# Autodesk Inventor assembly: WRO FE vehicle v4.1
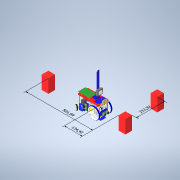
[picture p0: Inventor's stored thumbnail of the model, 180x180]
Saved by Autodesk Inventor 2022.6 (Build 266554000, 554)
## iProperties
Created: 2024-10-12
Part Number: WRO FE vehicle v4.1
Document SubType Name: Assembly
Designer: Zhong
Author: Zhong
## Documents named in this file (41)
- C:\Users\Zhong\Desktop\SP\YR_3_SEM_1\WRO\Robot\vehicle v8.4\WRO FE vehicle v8.iam
- C:\Users\Zhong\Desktop\SP\YR_3_SEM_1\WRO\Robot\vehicle v8.4\rear wheel 86mm.ipt
- C:\Users\Zhong\Desktop\SP\YR_3_SEM_1\WRO\Robot\vehicle v8.4\dfifferential.ipt
- C:\Users\Zhong\Desktop\SP\YR_3_SEM_1\WRO\Robot\vehicle v8.4\rear shaft v2.ipt
- rear shaft.ipt
- C:\Users\Zhong\Desktop\SP\YR_3_SEM_1\WRO\Robot\vehicle v8.4\Bottom plate.ipt
- C:\Users\Zhong\Desktop\SP\YR_3_SEM_1\WRO\Robot\vehicle v8.4\motor_small.ipt
- C:\Users\Zhong\Desktop\SP\YR_3_SEM_1\WRO\Robot\vehicle v8.4\driver gear adapter v2.ipt
- C:\Users\Zhong\Desktop\SP\YR_3_SEM_1\WRO\Robot\vehicle v8.4\DC+bearing mount.ipt
- C:\Users\Zhong\Desktop\SP\YR_3_SEM_1\WRO\Robot\vehicle v8.4\new battery.ipt
- C:\Users\Zhong\Desktop\SP\YR_3_SEM_1\WRO\Robot\vehicle v8.4\servo motor HS-7955TG.iam
- C:\Users\Zhong\Desktop\SP\YR_3_SEM_1\WRO\Robot\vehicle v8.4\US-015.ipt
- C:\Users\Zhong\Desktop\SP\YR_3_SEM_1\WRO\Robot\vehicle v8.4\stand M3-L30.ipt
- C:\Users\Zhong\Desktop\SP\YR_3_SEM_1\WRO\Robot\vehicle v8.4\Top plate.ipt
- C:\Users\Zhong\Desktop\SP\YR_3_SEM_1\WRO\Robot\vehicle v8.4\stand M3-L10.ipt
- C:\Users\Zhong\Desktop\SP\YR_3_SEM_1\WRO\Robot\vehicle v8.4\raspberry pi.ipt
- C:\Users\Zhong\Desktop\SP\YR_3_SEM_1\WRO\Robot\vehicle v8.4\Vertical Ultrasonic Sensor Mount.ipt
- C:\Users\Zhong\Desktop\SP\YR_3_SEM_1\WRO\Robot\vehicle v8.4\ultrasonic and headlight mount.ipt
- C:\Users\Zhong\Desktop\SP\YR_3_SEM_1\WRO\Robot\vehicle v8.4\MainLink.ipt
- C:\Users\Zhong\Desktop\SP\YR_3_SEM_1\WRO\Robot\vehicle v8.4\ActuatorLink.ipt
- C:\Users\Zhong\Desktop\SP\YR_3_SEM_1\WRO\Robot\vehicle v8.4\Battery Mount V2.ipt
- C:\Users\Zhong\Desktop\SP\YR_3_SEM_1\WRO\Robot\vehicle v8.4\Wheel_Pivot.ipt
- C:\Users\Zhong\Desktop\SP\YR_3_SEM_1\WRO\Robot\vehicle v8.4\LM2596 Buck Converter.ipt
- C:\Users\Zhong\Desktop\SP\YR_3_SEM_1\WRO\Robot\vehicle v8.4\LED Light.ipt
- C:\Users\Zhong\Desktop\SP\YR_3_SEM_1\WRO\Robot\vehicle v8.4\front wheel v2.ipt
- C:\Users\Zhong\Desktop\SP\YR_3_SEM_1\WRO\Robot\vehicle v8.4\front wheel mount.ipt
- C:\Users\Zhong\Desktop\SP\YR_3_SEM_1\WRO\Robot\vehicle v8.4\camera mount+HMC angled.ipt
- C:\Users\Zhong\Desktop\SP\YR_3_SEM_1\WRO\Robot\vehicle v8.4\Obstacle.ipt
- C:\Users\Zhong\Desktop\SP\YR_3_SEM_1\WRO\Robot\vehicle v8.4\cam vision.ipt
- C:\Users\Zhong\Desktop\SP\YR_3_SEM_1\WRO\Robot\vehicle v8.4\stand M3-L5.ipt
- C:\Users\Zhong\Desktop\SP\YR_3_SEM_1\WRO\Robot\vehicle v8.4\Servo steering actuator.ipt
- C:\Users\Zhong\Desktop\SP\YR_3_SEM_1\WRO\Robot\vehicle v8.4\Servo mount.ipt
- C:\Users\Zhong\Desktop\SP\YR_3_SEM_1\WRO\Robot\vehicle v8.4\Servo mount Right.ipt
- C:\Users\Zhong\Desktop\SP\YR_3_SEM_1\WRO\Robot\vehicle v8.4\Servo steering actuator v2.ipt
- C:\Users\Zhong\Desktop\SP\YR_3_SEM_1\WRO\Robot\vehicle v8.4\Vertical TOF mount.ipt
- C:\Users\Zhong\Desktop\SP\YR_3_SEM_1\WRO\Robot\vehicle v8.4\stand M3-L7.ipt
- C:\Users\Zhong\Desktop\SP\YR_3_SEM_1\WRO\Robot\vehicle v8.4\camera mount.ipt
- C:\Users\Zhong\Desktop\SP\YR_3_SEM_1\WRO\Robot\vehicle v8.4\IMU mount.ipt
- C:\Users\Zhong\Desktop\SP\YR_3_SEM_1\WRO\Robot\vehicle v8.4\front TOF mount.ipt
- C:\Users\Zhong\Desktop\SP\YR_3_SEM_1\WRO\Robot\vehicle v8.4\camera+light+IMU.ipt
- C:\Users\Zhong\Desktop\SP\YR_3_SEM_1\WRO\Robot\vehicle v8.4\cam mount prototype.ipt
## Components (74 placed, 39 different names)
1. rear wheel 86mm:1 — Tangent:2, Insert:4, Symmetry:1
2. rear wheel 86mm:2 — Tangent:1, Insert:2, Symmetry:1
3. dfifferential:1 — Angle:4, Insert:1, Insert:3
4. rear shaft:1 — Insert:3, Insert:4, Mate:20
5. rear shaft:2 — Insert:1, Insert:2
6. Bottom plate:1 — Flush:1, Tangent:3, Angle:5, Flush:2, Mate:1, Mate:2, Mate:3, Insert:17, Insert:18, Mate:95, Insert:21, Insert:22, Insert:23, Insert:24, Mate:108, Insert:71, Insert:72, Mate:110, Insert:75, Mate:112, Insert:77, Insert:78, Mate:113, Insert:87, Insert:89, Insert:94, Insert:95, Insert:96, Insert:97, Insert:98, Mate:116, Mate:117, Insert:101, Flush:116, Mate:124, Flush:117, Mate:125
7. motor_small:1 — Tangent:3, Flush:2, Insert:14, Insert:123
8. driver gear adapter v2:1 — Insert:123
9. DC+bearing mount:1 — Mate:1, Mate:2, Mate:3, Mate:20, Insert:14
10. new battery:1 — Mate:119, Mate:120, Mate:121
11. servo motor HS-7955TG:1 [sub-assembly] — Mate:95, Mate:110, Mate:113, Insert:80, Mate:114, Insert:85, Insert:86, Insert:92, Insert:93, Insert:126
12. US-015:1 — Insert:15, Insert:16
13. Top plate:1 — Insert:49, Insert:50, Insert:55, Insert:56, Insert:57, Insert:59, Insert:60, Insert:79, Insert:102, Insert:103, Insert:108, Insert:109, Mate:123, Insert:119, Insert:120
14. raspberry pi:1 — Insert:45, Insert:46, Insert:47, Insert:48
15. Vertical Ultrasonic Sensor Mount:1 — Mate:64, Mate:65, Mate:66, Insert:21, Insert:22
16. Vertical Ultrasonic Sensor Mount:2 — Mate:61, Mate:62, Mate:63, Insert:23, Insert:24
17. US-015:2 — Mate:64, Mate:65, Mate:66
18. US-015:3 — Mate:61, Mate:62, Mate:63
19. ultrasonic and headlight mount:1 — Insert:15, Insert:16, Insert:17, Insert:18
20. MainLink:1 — Mate:102, Insert:77, Insert:78, Angle:6
21. ActuatorLink:1 — Mate:97, Mate:99, Angle:6, Tangent:6, Insert:99, Insert:100, Tangent:7
22. Wheel_Pivot:1 — Mate:97, Insert:82, Insert:97, Insert:100
23. Wheel_Pivot:2 — Mate:99, Mate:102, Insert:81, Insert:98, Insert:99
24. LED Light:1 — Mate:122, Insert:135
25. front wheel v2:1 — Tangent:4, Insert:83, Flush:115
26. front wheel v2:2 — Flush:112, Tangent:5, Insert:84
27. front wheel mount:1 — Flush:112, Mate:112, Insert:81, Insert:84
28. stand M3-L10:13 — Insert:117
29. stand M3-L10:14 — Insert:44, Insert:116
30. stand M3-L10:15 — Insert:118
31. stand M3-L10:16 — Insert:112, Insert:115
32. Obstacle:1 — Mate:107, Mate:108, Flush:118, Flush:119
33. cam vision:1 — Insert:44, Insert:112, Insert:127, Insert:128
34. stand M3-L10:17 — Insert:48
35. stand M3-L10:18 — Insert:46, Insert:50
36. stand M3-L10:19 — Insert:47
37. stand M3-L10:20 — Insert:45, Insert:49
38. stand M3-L5:1 — Insert:56, Insert:113, Insert:129
39. stand M3-L5:2
40. stand M3-L5:3
41. stand M3-L5:4 — Insert:55, Insert:114, Insert:130
42. stand M3-L5:5 — Insert:79
43. stand M3-L5:6 — Insert:59, Insert:61
44. stand M3-L5:7 — Insert:60
45. stand M3-L5:8 — Insert:57, Insert:62
46. LM2596 Buck Converter:1 — Insert:61, Insert:62
47. stand M3-L30:1 — Insert:66, Insert:122
48. stand M3-L30:2 — Insert:66
49. stand M3-L30:3 — Insert:65, Insert:121
50. stand M3-L30:4 — Insert:65, Insert:72
51. stand M3-L30:5 — Insert:64, Insert:71
52. stand M3-L30:6 — Insert:64, Insert:104
53. stand M3-L30:7 — Insert:63, Insert:105
54. stand M3-L30:8 — Insert:63, Insert:75
55. Servo steering actuator:1 — Tangent:6, Insert:80
56. front wheel mount:2 — Insert:82, Insert:83, Flush:115
57. Servo mount:1 — Mate:114, Insert:85, Insert:86, Insert:87, Insert:89, Insert:101
58. Servo mount Right:1 — Insert:92, Insert:93, Insert:94, Insert:95, Insert:96
59. Servo steering actuator v2:1 — Mate:116, Insert:126, Tangent:7
60. Vertical TOF mount:1 — Mate:117, Flush:116
61. Battery Mount V2:1 — Insert:102, Insert:103, Mate:119, Mate:120, Mate:121
62. stand M3-L7:1 — Insert:104, Insert:108
63. stand M3-L7:2 — Insert:105, Insert:109
64. Obstacle:2 — Flush:119
65. camera mount+HMC angled:1 — Mate:122, Insert:113, Insert:114, Insert:135, Insert:136, Insert:137
66. camera mount:1 — Mate:123, Insert:115, Insert:116, Insert:117, Insert:118, Insert:119, Insert:120
67. stand M3-L5:9 — Insert:122
68. stand M3-L5:10 — Insert:121
69. IMU mount:1 — Insert:136, Insert:137
70. front TOF mount:1 — Mate:125
71. camera+light+IMU:1 — Insert:127, Insert:128, Insert:129, Insert:130
72. Obstacle:3 — Flush:118
73. cam mount prototype:1
74. Vertical TOF mount:2 — Mate:124, Flush:117
## Relationships (131: Insert 82, Mate 29, Flush 8, Tangent 7, Angle 4, Symmetry 1)
- Tangent:1: rear wheel 86mm:2
- Angle:2 (0 deg)
- Tangent:2: rear wheel 86mm:1
- Angle:4 (0 deg): dfifferential:1
- Insert:1: dfifferential:1 ↔ rear shaft:2
- Insert:2 (-2 mm): rear wheel 86mm:2 ↔ rear shaft:2
- Insert:3: dfifferential:1 ↔ rear shaft:1
- Insert:4 (-2 mm): rear wheel 86mm:1 ↔ rear shaft:1
- Flush:1: Bottom plate:1
- Symmetry:1: rear wheel 86mm:1 ↔ rear wheel 86mm:2
- Tangent:3 (6 mm): Bottom plate:1 ↔ motor_small:1
- Angle:5 (180 deg): Bottom plate:1
- Flush:2: Bottom plate:1 ↔ motor_small:1
- Mate:1: Bottom plate:1 ↔ DC+bearing mount:1
- Mate:2: Bottom plate:1 ↔ DC+bearing mount:1
- Mate:3: Bottom plate:1 ↔ DC+bearing mount:1
- Mate:20: rear shaft:1 ↔ DC+bearing mount:1
- Mate:61: Vertical Ultrasonic Sensor Mount:2 ↔ US-015:3
- Mate:62: Vertical Ultrasonic Sensor Mount:2 ↔ US-015:3
- Mate:63: Vertical Ultrasonic Sensor Mount:2 ↔ US-015:3
- Mate:64: Vertical Ultrasonic Sensor Mount:1 ↔ US-015:2
- Mate:65: Vertical Ultrasonic Sensor Mount:1 ↔ US-015:2
- Mate:66: Vertical Ultrasonic Sensor Mount:1 ↔ US-015:2
- Insert:14: motor_small:1 ↔ DC+bearing mount:1
- Insert:15: US-015:1 ↔ ultrasonic and headlight mount:1
- Insert:16: US-015:1 ↔ ultrasonic and headlight mount:1
- Insert:17: Bottom plate:1 ↔ ultrasonic and headlight mount:1
- Insert:18: Bottom plate:1 ↔ ultrasonic and headlight mount:1
- Mate:95: Bottom plate:1 ↔ servo motor HS-7955TG:1
- Mate:97: ActuatorLink:1 ↔ Wheel_Pivot:1
- Mate:99: ActuatorLink:1 ↔ Wheel_Pivot:2
- Mate:102: MainLink:1 ↔ Wheel_Pivot:2
- Insert:21: Bottom plate:1 ↔ Vertical Ultrasonic Sensor Mount:1
- Insert:22: Bottom plate:1 ↔ Vertical Ultrasonic Sensor Mount:1
- Insert:23: Bottom plate:1 ↔ Vertical Ultrasonic Sensor Mount:2
- Insert:24: Bottom plate:1 ↔ Vertical Ultrasonic Sensor Mount:2
- Flush:112: front wheel v2:2 ↔ front wheel mount:1
- Mate:107: Obstacle:1
- Mate:108: Bottom plate:1 ↔ Obstacle:1
- Insert:44: stand M3-L10:14 ↔ cam vision:1
- Insert:45: raspberry pi:1 ↔ stand M3-L10:20
- Insert:46: raspberry pi:1 ↔ stand M3-L10:18
- Insert:47: raspberry pi:1 ↔ stand M3-L10:19
- Insert:48: raspberry pi:1 ↔ stand M3-L10:17
- Insert:49: Top plate:1 ↔ stand M3-L10:20
- Insert:50: Top plate:1 ↔ stand M3-L10:18
- Insert:55: Top plate:1 ↔ stand M3-L5:4
- Insert:56: Top plate:1 ↔ stand M3-L5:1
- Insert:57: Top plate:1 ↔ stand M3-L5:8
- Insert:59: Top plate:1 ↔ stand M3-L5:6
- Insert:60: Top plate:1 ↔ stand M3-L5:7
- Insert:61: stand M3-L5:6 ↔ LM2596 Buck Converter:1
- Insert:62: stand M3-L5:8 ↔ LM2596 Buck Converter:1
- Insert:63: stand M3-L30:7 ↔ stand M3-L30:8
- Insert:64: stand M3-L30:5 ↔ stand M3-L30:6
- Insert:65: stand M3-L30:3 ↔ stand M3-L30:4
- Insert:66: stand M3-L30:1 ↔ stand M3-L30:2
- Insert:71: Bottom plate:1 ↔ stand M3-L30:5
- Insert:72: Bottom plate:1 ↔ stand M3-L30:4
- Mate:110: Bottom plate:1 ↔ servo motor HS-7955TG:1
- Insert:75: Bottom plate:1 ↔ stand M3-L30:8
- Tangent:4: front wheel v2:1
- Mate:112: Bottom plate:1 ↔ front wheel mount:1
- Tangent:5: front wheel v2:2
- Insert:77: Bottom plate:1 ↔ MainLink:1
- Insert:78: Bottom plate:1 ↔ MainLink:1
- Mate:113 (8 mm): Bottom plate:1 ↔ servo motor HS-7955TG:1
- Insert:79: Top plate:1 ↔ stand M3-L5:5
- Angle:6 (0 deg): MainLink:1 ↔ ActuatorLink:1
- Tangent:6: ActuatorLink:1 ↔ Servo steering actuator:1
- Insert:80 (2 mm): servo motor HS-7955TG:1 ↔ Servo steering actuator:1
- Insert:81: Wheel_Pivot:2 ↔ front wheel mount:1
- Insert:82: Wheel_Pivot:1 ↔ front wheel mount:2
- Insert:83 (1 mm): front wheel v2:1 ↔ front wheel mount:2
- Flush:115: front wheel v2:1 ↔ front wheel mount:2
- Insert:84: front wheel v2:2 ↔ front wheel mount:1
- Mate:114: servo motor HS-7955TG:1 ↔ Servo mount:1
- Insert:85: servo motor HS-7955TG:1 ↔ Servo mount:1
- Insert:86: servo motor HS-7955TG:1 ↔ Servo mount:1
- Insert:87: Bottom plate:1 ↔ Servo mount:1
- Insert:89: Bottom plate:1 ↔ Servo mount:1
- Insert:92: servo motor HS-7955TG:1 ↔ Servo mount Right:1
- Insert:93: servo motor HS-7955TG:1 ↔ Servo mount Right:1
- Insert:94: Bottom plate:1 ↔ Servo mount Right:1
- Insert:95: Bottom plate:1 ↔ Servo mount Right:1
- Insert:96: Bottom plate:1 ↔ Servo mount Right:1
- Insert:97: Bottom plate:1 ↔ Wheel_Pivot:1
- Insert:98: Bottom plate:1 ↔ Wheel_Pivot:2
- Mate:116: Bottom plate:1 ↔ Servo steering actuator v2:1
- Mate:117: Bottom plate:1 ↔ Vertical TOF mount:1
- Insert:99: ActuatorLink:1 ↔ Wheel_Pivot:2
- Insert:100: ActuatorLink:1 ↔ Wheel_Pivot:1
- Insert:101: Bottom plate:1 ↔ Servo mount:1
- Insert:102: Top plate:1 ↔ Battery Mount V2:1
- Insert:103: Top plate:1 ↔ Battery Mount V2:1
- Mate:119: new battery:1 ↔ Battery Mount V2:1
- Mate:120: new battery:1 ↔ Battery Mount V2:1
- Mate:121: new battery:1 ↔ Battery Mount V2:1
- Insert:104: stand M3-L30:6 ↔ stand M3-L7:1
- Insert:105: stand M3-L30:7 ↔ stand M3-L7:2
- Insert:108: Top plate:1 ↔ stand M3-L7:1
- Insert:109: Top plate:1 ↔ stand M3-L7:2
- Insert:112: stand M3-L10:16 ↔ cam vision:1
- Mate:122: LED Light:1 ↔ camera mount+HMC angled:1
- Insert:113: stand M3-L5:1 ↔ camera mount+HMC angled:1
- Insert:114: stand M3-L5:4 ↔ camera mount+HMC angled:1
- Mate:123: Top plate:1 ↔ camera mount:1
- Insert:115: stand M3-L10:16 ↔ camera mount:1
- Insert:116: stand M3-L10:14 ↔ camera mount:1
- Insert:117: stand M3-L10:13 ↔ camera mount:1
- Insert:118: stand M3-L10:15 ↔ camera mount:1
- Insert:119: Top plate:1 ↔ camera mount:1
- Insert:120: Top plate:1 ↔ camera mount:1
- Insert:121: stand M3-L30:3 ↔ stand M3-L5:10
- Insert:122: stand M3-L30:1 ↔ stand M3-L5:9
- Insert:123 (-4 mm): motor_small:1 ↔ driver gear adapter v2:1
- Insert:126 (1 mm): servo motor HS-7955TG:1 ↔ Servo steering actuator v2:1
- Tangent:7: ActuatorLink:1 ↔ Servo steering actuator v2:1
- Insert:127: cam vision:1 ↔ camera+light+IMU:1
- Insert:128: cam vision:1 ↔ camera+light+IMU:1
- Insert:129: stand M3-L5:1 ↔ camera+light+IMU:1
- Insert:130: stand M3-L5:4 ↔ camera+light+IMU:1
- Insert:135: LED Light:1 ↔ camera mount+HMC angled:1
- Flush:116: Bottom plate:1 ↔ Vertical TOF mount:1
- Mate:124: Bottom plate:1 ↔ Vertical TOF mount:2
- Flush:117: Bottom plate:1 ↔ Vertical TOF mount:2
- Mate:125: Bottom plate:1 ↔ front TOF mount:1
- Insert:136: camera mount+HMC angled:1 ↔ IMU mount:1
- Insert:137: camera mount+HMC angled:1 ↔ IMU mount:1
- Flush:118: Obstacle:1 ↔ Obstacle:3
- Flush:119: Obstacle:1 ↔ Obstacle:2
